# Autodesk Inventor assembly: Assembly_ETL_v0
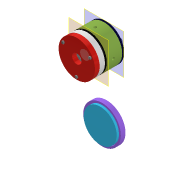
[picture p0: Inventor's stored thumbnail of the model, 180x180]
Saved by Autodesk Inventor 2022 (Build 260153000, 153)
## iProperties
Created: 2021-12-31
Part Number: Assembly_ETL_v0
Document SubType Name: Assembly
Designer: diederichbenedict
Mass: 22.6345 g
Surface Area: 191.935 cm^2
Volume: 22.6345 cm^3
Density: 1 g/cm^3
Author: diederichbenedict
## Documents named in this file (14)
- C:\Users\diederichbenedict\Dropbox\Dokumente\Promotion\PROJECTS\UC2\02_CAD\INVENTOR\uc2_v3\Assembly_ETL_v0.iam
- C:\Users\diederichbenedict\Dropbox\Dokumente\Promotion\PROJECTS\UC2\02_CAD\INVENTOR\uc2_v3\50_ETL_Membrane_v0.ipt
- C:\Users\diederichbenedict\Dropbox\Dokumente\Promotion\PROJECTS\UC2\02_CAD\INVENTOR\uc2_v3\50_ETL_28by_coil.ipt
- C:\Users\diederichbenedict\Dropbox\Dokumente\Promotion\PROJECTS\UC2\02_CAD\INVENTOR\uc2_v3\00_Ringmagnet_10x5x3mm.ipt
- C:\Users\diederichbenedict\Dropbox\Dokumente\Promotion\PROJECTS\UC2\02_CAD\INVENTOR\uc2_v3\50_ETL_Base_v0.ipt
- C:\Users\diederichbenedict\Dropbox\Dokumente\Promotion\PROJECTS\UC2\02_CAD\INVENTOR\uc2_v3\50_ETL_Lid_v0.ipt
- C:\Users\diederichbenedict\Dropbox\Dokumente\Promotion\PROJECTS\UC2\02_CAD\INVENTOR\uc2_v3\00_coverglass_10mm.ipt
- C:\Users\diederichbenedict\Dropbox\Dokumente\Promotion\PROJECTS\UC2\02_CAD\INVENTOR\uc2_v3\00_coverglass_25mm.ipt
- C:\Users\diederichbenedict\Dropbox\Dokumente\Promotion\PROJECTS\UC2\02_CAD\INVENTOR\uc2_v3\50_ETL_Spring_v0.ipt
- C:\Users\diederichbenedict\Documents\Inventor\Content Center Files\R2022\de-DE\DIN 912\DIN 912 - M3 x 0.5 x 30 x 18.ipt
- C:\Users\diederichbenedict\Dropbox\Dokumente\Promotion\PROJECTS\UC2\02_CAD\INVENTOR\uc2_v3\50_ETL_Motionpart1_v0.ipt
- C:\Users\diederichbenedict\Dropbox\Dokumente\Promotion\PROJECTS\UC2\02_CAD\INVENTOR\uc2_v3\50_ETL_Base_layer1_v0.ipt
- C:\Users\diederichbenedict\Dropbox\Dokumente\Promotion\PROJECTS\UC2\02_CAD\INVENTOR\uc2_v3\50_Assembly_ETL_Mould.ipt
- C:\Users\diederichbenedict\Dropbox\Dokumente\Promotion\PROJECTS\UC2\02_CAD\INVENTOR\uc2_v3\50_Assembly_ETL_Mould.iam
## Components (16 placed, 12 different names)
1. 50_ETL_Membrane_v0:1 — Einfügen:7, Einfügen:11
2. 00_Ringmagnet_10x5x3mm:1 — Einfügen:7
3. 50_ETL_Lid_v0:1 — Einfügen:3, Fluchtend:8
4. 00_coverglass_10mm:1
5. 00_coverglass_25mm:1 — Einfügen:3
6. DIN 912 - ersetzt durch DIN EN ISO 4762 M3 x 30:1
7. DIN 912 - ersetzt durch DIN EN ISO 4762 M3 x 30:2
8. DIN 912 - ersetzt durch DIN EN ISO 4762 M3 x 30:3
9. 50_ETL_Base_layer1_v0:1 — Fluchtend:8, Einfügen:4, Passend:1
10. 50_Assembly_ETL_Mould:1
11. 50_Assembly_ETL_Mould:2 [sub-assembly]
12. 50_ETL_Spring_v0:3 — Einfügen:4, Passend:1, Einfügen:12
13. 50_ETL_Motionpart1_v0:1 — Einfügen:11
14. 50_ETL_Spring_v0:4 — Einfügen:13
15. 50_ETL_Base_v0:1 — Einfügen:12, Einfügen:13, Einfügen:14
16. 50_ETL_28by_coil:3 — Einfügen:14
## Relationships (9: Insert 7, Flush 1, Mate 1)
- Einfügen:3 [Insert]: 50_ETL_Lid_v0:1 ↔ 00_coverglass_25mm:1
- Fluchtend:8 [Flush]: 50_ETL_Lid_v0:1 ↔ 50_ETL_Base_layer1_v0:1
- Einfügen:4 [Insert]: 50_ETL_Base_layer1_v0:1 ↔ 50_ETL_Spring_v0:3
- Passend:1 [Mate]: 50_ETL_Base_layer1_v0:1 ↔ 50_ETL_Spring_v0:3
- Einfügen:7 [Insert]: 50_ETL_Membrane_v0:1 ↔ 00_Ringmagnet_10x5x3mm:1
- Einfügen:11 [Insert]: 50_ETL_Membrane_v0:1 ↔ 50_ETL_Motionpart1_v0:1
- Einfügen:12 [Insert]: 50_ETL_Spring_v0:3 ↔ 50_ETL_Base_v0:1
- Einfügen:13 [Insert]: 50_ETL_Spring_v0:4 ↔ 50_ETL_Base_v0:1
- Einfügen:14 [Insert]: 50_ETL_Base_v0:1 ↔ 50_ETL_28by_coil:3
